# Autodesk Inventor assembly: Drive 60V Transmission
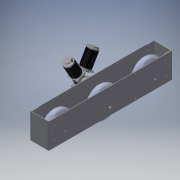
[picture p0: Inventor's stored thumbnail of the model, 180x180]
Saved by Autodesk Inventor 2017 (Build 210142000, 142)
## iProperties
Created: 2019-03-05
Part Number: Drive 60V Transmission
Document SubType Name: Assembly
Designer: S346553810
Author: S346553810
## Documents named in this file (5)
- \\ad.ocdsb.ca\studenthome\3\S338674153\FRC 2020\FullRobotRefactor\ModularDriveTrain\Drive 60V Transmission.iam
- \\ad.ocdsb.ca\studenthome\3\S338674153\FRC 2020\FullRobotRefactor\ModularDriveTrain\EMR - Side Panel.ipt
- \\ad.ocdsb.ca\studenthome\3\S338674153\FRC 2020\FullRobotRefactor\ModularDriveTrain\8in wheel with double pulley.iam
- \\ad.ocdsb.ca\studenthome\3\S338674153\FRC 2020\FullRobotRefactor\ModularDriveTrain\EMR Drive Module End.ipt
- \\ad.ocdsb.ca\studenthome\3\S338674153\FRC 2020\FullRobotRefactor\GearBox\Gearbox_V_Rev4.iam
## Components (8 placed, 4 different names)
1. EMR - Side Panel:1 — Mate:4, Flush:1, Flush:2, Flush:5, Mate:10, Mate:18, Mate:19, Mate:20, Mate:21, Mate:22
2. EMR - Side Panel:2 — Mate:7, Mate:8, Flush:3, Mate:9, Flush:4, Flush:6, Mate:14
3. 8in wheel with double pulley:1 [sub-assembly] — Mate:8, Flush:8
4. 8in wheel with double pulley:2 [sub-assembly] — Mate:7, Flush:7
5. 8in wheel with double pulley:3 [sub-assembly] — Mate:14, Flush:7, Flush:8, Mate:18
6. EMR Drive Module End:1 — Mate:4, Flush:1, Flush:2, Flush:3, Mate:9
7. EMR Drive Module End:2 — Flush:4, Flush:5, Mate:10, Flush:6
8. Gearbox_V_Rev4:1 [sub-assembly] — Mate:19, Mate:20, Mate:21, Mate:22
## Relationships (19: Mate 11, Flush 8)
- Mate:4: EMR - Side Panel:1 ↔ EMR Drive Module End:1
- Flush:1: EMR - Side Panel:1 ↔ EMR Drive Module End:1
- Flush:2: EMR - Side Panel:1 ↔ EMR Drive Module End:1
- Mate:7: EMR - Side Panel:2 ↔ 8in wheel with double pulley:2
- Mate:8: EMR - Side Panel:2 ↔ 8in wheel with double pulley:1
- Flush:3: EMR - Side Panel:2 ↔ EMR Drive Module End:1
- Mate:9: EMR - Side Panel:2 ↔ EMR Drive Module End:1
- Flush:4: EMR - Side Panel:2 ↔ EMR Drive Module End:2
- Flush:5: EMR - Side Panel:1 ↔ EMR Drive Module End:2
- Mate:10: EMR - Side Panel:1 ↔ EMR Drive Module End:2
- Flush:6: EMR - Side Panel:2 ↔ EMR Drive Module End:2
- Mate:14: EMR - Side Panel:2 ↔ 8in wheel with double pulley:3
- Flush:7: 8in wheel with double pulley:2 ↔ 8in wheel with double pulley:3
- Flush:8: 8in wheel with double pulley:1 ↔ 8in wheel with double pulley:3
- Mate:18: EMR - Side Panel:1 ↔ 8in wheel with double pulley:3
- Mate:19: EMR - Side Panel:1 ↔ Gearbox_V_Rev4:1
- Mate:20: EMR - Side Panel:1 ↔ Gearbox_V_Rev4:1
- Mate:21: EMR - Side Panel:1 ↔ Gearbox_V_Rev4:1
- Mate:22: EMR - Side Panel:1 ↔ Gearbox_V_Rev4:1
